# Autodesk Inventor assembly: 組合檔
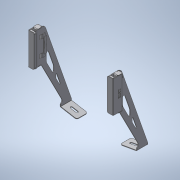
[picture p0: Inventor's stored thumbnail of the model, 180x180]
Saved by Autodesk Inventor 2020 (Build 240168000, 168)
## iProperties
Created: 2015-11-28
Part Number: 組合檔
Document SubType Name: Assembly
Designer: 設計製圖
Author: 設計製圖
## Documents named in this file (24)
- D:\資料庫\設計-3D Project\【May club 】\得利卡-車頂燈架\模型、圖面\車頂燈架長-組合(白鐵).iam
- D:\資料庫\設計-3D Project\【May club 】\得利卡-車頂燈架\模型、圖面\現成品-組裝零件\概-膠條.ipt
- D:\資料庫\設計-3D Project\【May club 】\得利卡-車頂燈架\模型、圖面\現成品-組裝零件\概-泡棉墊(1).ipt
- D:\資料庫\設計-3D Project\【May club 】\得利卡-車頂燈架\模型、圖面\現成品-組裝零件\概-泡棉墊(3).ipt
- D:\資料庫\設計-3D Project\【 鐵蹄 】\------鐵蹄工廠素材------ -\拉帽-M8.ipt
- D:\資料庫\設計-3D Project\【May club 】\得利卡-車頂燈架\模型、圖面\白鐵-焊接組件-1.ipt
- D:\資料庫\設計-3D Project\【May club 】\得利卡-車頂燈架\模型、圖面\白鐵-焊接組件-3.ipt
- D:\資料庫\設計-3D Project\【May club 】\得利卡-車頂燈架\模型、圖面\現成品-組裝零件\概-泡棉墊(2).ipt
- D:\資料庫\設計-3D Project\【May club 】\得利卡-車頂燈架\模型、圖面\白鐵-焊接組件-2.ipt
- D:\資料庫\設計-3D Project\材料庫\【螺絲】\止付螺絲\止付螺絲-M8-20.ipt
- D:\資料庫\設計-3D Project\【May club 】\得利卡-車頂燈架\模型、圖面\車身圖.ipt
- D:\資料庫\設計-3D Project\【May club 】\得利卡-車頂燈架\模型、圖面\白鐵-吊架組件-ㄇ槽.ipt
- D:\資料庫\設計-3D Project\【May club 】\得利卡-車頂燈架\模型、圖面\白鐵-吊架-長(R).ipt
- D:\資料庫\設計-3D Project\【May club 】\得利卡-車頂燈架\模型、圖面\白鐵-吊架組件-ㄇ槽_MIR.ipt
- D:\資料庫\設計-3D Project\【May club 】\得利卡-車頂燈架\模型、圖面\白鐵-吊架-長(L)_MIR.ipt
- D:\資料庫\設計-3D Project\【May club 】\得利卡-車頂燈架\模型、圖面\白鐵-焊接組件-1_MIR.ipt
- D:\資料庫\設計-3D Project\【May club 】\得利卡-車頂燈架\模型、圖面\白鐵-焊接組件-2_MIR.ipt
- D:\資料庫\設計-3D Project\【May club 】\得利卡-車頂燈架\模型、圖面\白鐵-焊接組件-3_MIR.ipt
- D:\資料庫\設計-3D Project\【 鐵蹄 】\------鐵蹄工廠素材------ -\拉帽-M8_MIR1.ipt
- D:\資料庫\設計-3D Project\【May club 】\得利卡-車頂燈架\模型、圖面\現成品-組裝零件\概-泡棉墊(2)_MIR3.ipt
- D:\資料庫\設計-3D Project\【May club 】\得利卡-車頂燈架\模型、圖面\現成品-組裝零件\概-膠條_MIR3.ipt
- D:\資料庫\設計-3D Project\【May club 】\得利卡-車頂燈架\模型、圖面\現成品-組裝零件\概-泡棉墊(1)_MIR3.ipt
- D:\資料庫\設計-3D Project\【May club 】\得利卡-車頂燈架\模型、圖面\現成品-組裝零件\概-泡棉墊(3)_MIR3.ipt
- D:\資料庫\設計-3D Project\材料庫\【螺絲】\止付螺絲\止付螺絲-M8-20_MIR1.ipt
## Components (27 placed, 23 different names)
1. 車身圖:1 — 貼合:33
2. 白鐵-吊架組件-ㄇ槽:1 — 貼合:6, 齊平:2, 齊平:3, 貼合:8, 齊平:4, 貼合:17, 貼合:18, 貼合:24, 貼合:35, 貼合:36, 貼合:37, 貼合:38, 齊平:13
3. 白鐵-吊架-長(R):1 — 貼合:3, 貼合:4, 齊平:1, 貼合:18, 貼合:23, 貼合:25, 貼合:26, 貼合:28, 齊平:9, 齊平:10, 貼合:33, 齊平:14
4. 白鐵-焊接組件-1:1 — 貼合:29, 貼合:30, 齊平:11
5. 白鐵-焊接組件-2:1 — 貼合:28, 齊平:9, 齊平:10, 貼合:29, 貼合:30, 齊平:11
6. 白鐵-焊接組件-3:1 — 貼合:23, 貼合:24, 貼合:25, 貼合:26, 貼合:27, 齊平:7, 齊平:8, 齊平:13
7. 拉帽-M8:1 — 齊平:6, 貼合:15, 貼合:17, 貼合:31, 貼合:35, 貼合:37
8. 拉帽-M8:2 — 齊平:6, 貼合:15, 貼合:32, 貼合:36, 貼合:38
9. 白鐵-吊架組件-ㄇ槽_MIR:1 — 貼合:39, 齊平:16, 齊平:17, 貼合:42, 齊平:18, 貼合:44, 貼合:45, 貼合:46, 貼合:47, 齊平:20, 貼合:51
10. 白鐵-吊架-長(L)_MIR:1 — 貼合:39, 齊平:15, 貼合:40, 貼合:41, 貼合:49, 貼合:50, 貼合:52, 齊平:24, 貼合:56, 貼合:57, 貼合:60
11. 白鐵-焊接組件-1_MIR:1 — 齊平:23, 貼合:54, 貼合:55
12. 白鐵-焊接組件-2_MIR:1 — 齊平:23, 貼合:54, 貼合:55, 齊平:24, 貼合:56, 貼合:57
13. 白鐵-焊接組件-3_MIR:1 — 齊平:20, 貼合:49, 貼合:50, 貼合:51, 貼合:52, 齊平:21, 齊平:22, 貼合:53
14. 拉帽-M8_MIR1:1 — 貼合:45, 貼合:46, 貼合:48, 齊平:19, 貼合:58
15. 拉帽-M8_MIR1:2 — 貼合:47, 貼合:48, 齊平:19, 貼合:59
16. 概-泡棉墊(2)_MIR3:1 — 齊平:21, 齊平:22, 貼合:53
17. 概-膠條_MIR3:1 — 齊平:15, 貼合:40, 貼合:41
18. 概-泡棉墊(1)_MIR3:1 — 齊平:16, 齊平:17, 貼合:42, 貼合:43
19. 概-泡棉墊(3)_MIR3:1 — 齊平:18, 貼合:43, 貼合:44
20. 止付螺絲-M8-20_MIR1:1 — 貼合:58, 齊平:25
21. 止付螺絲-M8-20_MIR1:2 — 貼合:59, 齊平:25
22. 概-泡棉墊(2):1 — 貼合:27, 齊平:7, 齊平:8
23. 概-膠條:1 — 貼合:3, 貼合:4, 齊平:1
24. 概-泡棉墊(1):1 — 貼合:6, 齊平:2, 齊平:3, 貼合:9
25. 概-泡棉墊(3):1 — 貼合:8, 貼合:9, 齊平:4
26. 止付螺絲-M8-20:1 — 齊平:12, 貼合:31
27. 止付螺絲-M8-20:2 — 齊平:12, 貼合:32
## Relationships (69: Mate 45, Flush 24)
- 貼合:3 [Mate]: 白鐵-吊架-長(R):1 ↔ 概-膠條:1
- 貼合:4 [Mate]: 白鐵-吊架-長(R):1 ↔ 概-膠條:1
- 齊平:1 [Flush]: 白鐵-吊架-長(R):1 ↔ 概-膠條:1
- 貼合:6 [Mate]: 白鐵-吊架組件-ㄇ槽:1 ↔ 概-泡棉墊(1):1
- 齊平:2 [Flush]: 白鐵-吊架組件-ㄇ槽:1 ↔ 概-泡棉墊(1):1
- 齊平:3 [Flush]: 白鐵-吊架組件-ㄇ槽:1 ↔ 概-泡棉墊(1):1
- 貼合:8 [Mate]: 白鐵-吊架組件-ㄇ槽:1 ↔ 概-泡棉墊(3):1
- 貼合:9 [Mate]: 概-泡棉墊(1):1 ↔ 概-泡棉墊(3):1
- 齊平:4 [Flush]: 白鐵-吊架組件-ㄇ槽:1 ↔ 概-泡棉墊(3):1
- 齊平:6 [Flush]: 拉帽-M8:1 ↔ 拉帽-M8:2
- 貼合:15 [Mate]: 拉帽-M8:1 ↔ 拉帽-M8:2
- 貼合:17 [Mate]: 白鐵-吊架組件-ㄇ槽:1 ↔ 拉帽-M8:1
- 貼合:18 [Mate]: 白鐵-吊架組件-ㄇ槽:1 ↔ 白鐵-吊架-長(R):1
- 貼合:23 [Mate]: 白鐵-吊架-長(R):1 ↔ 白鐵-焊接組件-3:1
- 貼合:24 [Mate]: 白鐵-吊架組件-ㄇ槽:1 ↔ 白鐵-焊接組件-3:1
- 貼合:25 [Mate]: 白鐵-吊架-長(R):1 ↔ 白鐵-焊接組件-3:1
- 貼合:26 [Mate]: 白鐵-吊架-長(R):1 ↔ 白鐵-焊接組件-3:1
- 貼合:27 [Mate]: 白鐵-焊接組件-3:1 ↔ 概-泡棉墊(2):1
- 齊平:7 [Flush]: 白鐵-焊接組件-3:1 ↔ 概-泡棉墊(2):1
- 齊平:8 [Flush]: 白鐵-焊接組件-3:1 ↔ 概-泡棉墊(2):1
- 貼合:28 [Mate]: 白鐵-吊架-長(R):1 ↔ 白鐵-焊接組件-2:1
- 齊平:9 [Flush]: 白鐵-吊架-長(R):1 ↔ 白鐵-焊接組件-2:1
- 齊平:10 [Flush] (33 mm): 白鐵-吊架-長(R):1 ↔ 白鐵-焊接組件-2:1
- 貼合:29 [Mate]: 白鐵-焊接組件-1:1 ↔ 白鐵-焊接組件-2:1
- 貼合:30 [Mate]: 白鐵-焊接組件-1:1 ↔ 白鐵-焊接組件-2:1
- 齊平:11 [Flush]: 白鐵-焊接組件-1:1 ↔ 白鐵-焊接組件-2:1
- 齊平:12 [Flush]: 止付螺絲-M8-20:1 ↔ 止付螺絲-M8-20:2
- 貼合:31 [Mate]: 拉帽-M8:1 ↔ 止付螺絲-M8-20:1
- 貼合:32 [Mate]: 拉帽-M8:2 ↔ 止付螺絲-M8-20:2
- 貼合:33 [Mate]: 車身圖:1 ↔ 白鐵-吊架-長(R):1
- 貼合:35 [Mate]: 白鐵-吊架組件-ㄇ槽:1 ↔ 拉帽-M8:1
- 貼合:36 [Mate]: 白鐵-吊架組件-ㄇ槽:1 ↔ 拉帽-M8:2
- 貼合:37 [Mate]: 白鐵-吊架組件-ㄇ槽:1 ↔ 拉帽-M8:1
- 貼合:38 [Mate]: 白鐵-吊架組件-ㄇ槽:1 ↔ 拉帽-M8:2
- 齊平:13 [Flush]: 白鐵-吊架組件-ㄇ槽:1 ↔ 白鐵-焊接組件-3:1
- 齊平:14 [Flush] (150 mm): 白鐵-吊架-長(R):1
- 貼合:39 [Mate]: 白鐵-吊架組件-ㄇ槽_MIR:1 ↔ 白鐵-吊架-長(L)_MIR:1
- 齊平:15 [Flush]: 白鐵-吊架-長(L)_MIR:1 ↔ 概-膠條_MIR3:1
- 貼合:40 [Mate]: 白鐵-吊架-長(L)_MIR:1 ↔ 概-膠條_MIR3:1
- 貼合:41 [Mate]: 白鐵-吊架-長(L)_MIR:1 ↔ 概-膠條_MIR3:1
- 齊平:16 [Flush]: 白鐵-吊架組件-ㄇ槽_MIR:1 ↔ 概-泡棉墊(1)_MIR3:1
- 齊平:17 [Flush]: 白鐵-吊架組件-ㄇ槽_MIR:1 ↔ 概-泡棉墊(1)_MIR3:1
- 貼合:42 [Mate]: 白鐵-吊架組件-ㄇ槽_MIR:1 ↔ 概-泡棉墊(1)_MIR3:1
- 齊平:18 [Flush]: 白鐵-吊架組件-ㄇ槽_MIR:1 ↔ 概-泡棉墊(3)_MIR3:1
- 貼合:43 [Mate]: 概-泡棉墊(1)_MIR3:1 ↔ 概-泡棉墊(3)_MIR3:1
- 貼合:44 [Mate]: 白鐵-吊架組件-ㄇ槽_MIR:1 ↔ 概-泡棉墊(3)_MIR3:1
- 貼合:45 [Mate]: 白鐵-吊架組件-ㄇ槽_MIR:1 ↔ 拉帽-M8_MIR1:1
- 貼合:46 [Mate]: 白鐵-吊架組件-ㄇ槽_MIR:1 ↔ 拉帽-M8_MIR1:1
- 貼合:47 [Mate]: 白鐵-吊架組件-ㄇ槽_MIR:1 ↔ 拉帽-M8_MIR1:2
- 貼合:48 [Mate]: 拉帽-M8_MIR1:1 ↔ 拉帽-M8_MIR1:2
- 齊平:19 [Flush]: 拉帽-M8_MIR1:1 ↔ 拉帽-M8_MIR1:2
- 齊平:20 [Flush]: 白鐵-吊架組件-ㄇ槽_MIR:1 ↔ 白鐵-焊接組件-3_MIR:1
- 貼合:49 [Mate]: 白鐵-吊架-長(L)_MIR:1 ↔ 白鐵-焊接組件-3_MIR:1
- 貼合:50 [Mate]: 白鐵-吊架-長(L)_MIR:1 ↔ 白鐵-焊接組件-3_MIR:1
- 貼合:51 [Mate]: 白鐵-吊架組件-ㄇ槽_MIR:1 ↔ 白鐵-焊接組件-3_MIR:1
- 貼合:52 [Mate]: 白鐵-吊架-長(L)_MIR:1 ↔ 白鐵-焊接組件-3_MIR:1
- 齊平:21 [Flush]: 白鐵-焊接組件-3_MIR:1 ↔ 概-泡棉墊(2)_MIR3:1
- 齊平:22 [Flush]: 白鐵-焊接組件-3_MIR:1 ↔ 概-泡棉墊(2)_MIR3:1
- 貼合:53 [Mate]: 白鐵-焊接組件-3_MIR:1 ↔ 概-泡棉墊(2)_MIR3:1
- 齊平:23 [Flush]: 白鐵-焊接組件-1_MIR:1 ↔ 白鐵-焊接組件-2_MIR:1
- 貼合:54 [Mate]: 白鐵-焊接組件-1_MIR:1 ↔ 白鐵-焊接組件-2_MIR:1
- 貼合:55 [Mate]: 白鐵-焊接組件-1_MIR:1 ↔ 白鐵-焊接組件-2_MIR:1
- 齊平:24 [Flush] (33 mm): 白鐵-吊架-長(L)_MIR:1 ↔ 白鐵-焊接組件-2_MIR:1
- 貼合:56 [Mate]: 白鐵-吊架-長(L)_MIR:1 ↔ 白鐵-焊接組件-2_MIR:1
- 貼合:57 [Mate]: 白鐵-吊架-長(L)_MIR:1 ↔ 白鐵-焊接組件-2_MIR:1
- 貼合:58 [Mate]: 拉帽-M8_MIR1:1 ↔ 止付螺絲-M8-20_MIR1:1
- 貼合:59 [Mate]: 拉帽-M8_MIR1:2 ↔ 止付螺絲-M8-20_MIR1:2
- 齊平:25 [Flush]: 止付螺絲-M8-20_MIR1:1 ↔ 止付螺絲-M8-20_MIR1:2
- 貼合:60 [Mate] (150 mm): 白鐵-吊架-長(L)_MIR:1
